# Autodesk Inventor assembly: PoweredWheelAssembly
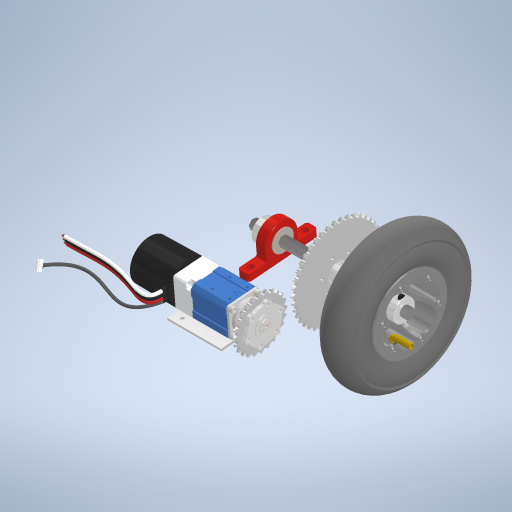
[picture p0: Inventor's stored thumbnail of the model, 512x512]
Saved by Autodesk Inventor 2023 (Build 270158000, 158)
## iProperties
Created: 2022-09-14
Part Number: PoweredWheelAssembly
Document SubType Name: Assembly
Designer: PC
Author: PC
## Documents named in this file (12)
- C:\Users\PC\Documents\PersonalCAD\ARCIGVC\IGVC-Robot\PoweredWheelAssembly.iam
- C:\Users\PC\Documents\PersonalCAD\ARCIGVC\IGVC-Robot\8inPneumatic.ipt
- C:\Users\PC\Documents\PersonalCAD\ARCIGVC\IGVC-Robot\2 Stage HD - CIM Sport.ipt
- C:\Users\PC\Documents\PersonalCAD\ARCIGVC\IGVC-Robot\am-4258 NEO Brushless Motor.ipt
- C:\Users\PC\Documents\PersonalCAD\ARCIGVC\IGVC-Robot\MotorMount.ipt
- C:\Users\PC\Documents\PersonalCAD\ARCIGVC\IGVC-Robot\24tSprocket35Series.ipt
- C:\Users\PC\Documents\PersonalCAD\ARCIGVC\IGVC-Robot\42tSprocket35Series.ipt
- C:\Users\PC\Documents\PersonalCAD\ARCIGVC\IGVC-Robot\Hex Hub .5In.ipt
- C:\Users\PC\Documents\PersonalCAD\ARCIGVC\IGVC-Robot\Bearing Housing.ipt
- C:\Users\PC\Documents\PersonalCAD\ARCIGVC\IGVC-Robot\HalfInHex Bearing.ipt
- C:\Users\PC\Documents\PersonalCAD\ARCIGVC\IGVC-Robot\9in-0.5inHexAxel.ipt
- C:\Users\PC\Documents\PersonalCAD\ARCIGVC\IGVC-Robot\am-1526 500Hex HD Collar Clamp.ipt
## Components (17 placed, 11 different names)
1. 8inPneumatic:1 — Mate:35
2. 2 Stage HD - CIM Sport:1
3. am-4258 NEO Brushless Motor:1
4. MotorMount:1 — Flush:6, Flush:7
5. 24tSprocket35Series:1
6. 42tSprocket35Series:1
7. Hex Hub .5In:1
8. Hex Hub .5In:2
9. Bearing Housing:1 — Flush:4, Mate:35
10. Bearing Housing:2 — Flush:4, Flush:5, Flush:6, Flush:7
11. HalfInHex Bearing:1
12. HalfInHex Bearing:2
13. HalfInHex Bearing:3
14. HalfInHex Bearing:4
15. 9in-0.5inHexAxel:1 — Flush:5
16. am-1526 500Hex HD Collar Clamp:1
17. am-1526 500Hex HD Collar Clamp:2
## Relationships (42: Mate 35, Flush 7)
- [Mate]: 2 Stage HD - CIM Sport:1 ↔ am-4258 NEO Brushless Motor:1
- [Mate]: 2 Stage HD - CIM Sport:1 ↔ am-4258 NEO Brushless Motor:1
- [Mate]: 2 Stage HD - CIM Sport:1 ↔ am-4258 NEO Brushless Motor:1
- [Mate]: 2 Stage HD - CIM Sport:1 ↔ MotorMount:1
- [Mate]: 2 Stage HD - CIM Sport:1 ↔ MotorMount:1
- [Mate]: 2 Stage HD - CIM Sport:1 ↔ MotorMount:1
- [Mate]: 24tSprocket35Series:1 ↔ Hex Hub .5In:2
- [Mate]: 24tSprocket35Series:1 ↔ Hex Hub .5In:2
- [Mate]: 24tSprocket35Series:1 ↔ Hex Hub .5In:2
- [Mate]: 2 Stage HD - CIM Sport:1 ↔ Hex Hub .5In:2
- [Flush]: 2 Stage HD - CIM Sport:1 ↔ Hex Hub .5In:2
- [Mate]: 42tSprocket35Series:1 ↔ Hex Hub .5In:1
- [Mate]: 42tSprocket35Series:1 ↔ Hex Hub .5In:1
- [Mate]: 42tSprocket35Series:1 ↔ Hex Hub .5In:1
- [Mate]: Bearing Housing:1 ↔ Bearing Housing:2
- [Mate]: Bearing Housing:1 ↔ HalfInHex Bearing:1
- [Mate]: Bearing Housing:1 ↔ HalfInHex Bearing:1
- [Mate]: Bearing Housing:1 ↔ HalfInHex Bearing:2
- [Mate]: Bearing Housing:1 ↔ HalfInHex Bearing:2
- [Mate]: Bearing Housing:2 ↔ HalfInHex Bearing:3
- [Mate]: Bearing Housing:2 ↔ HalfInHex Bearing:4
- [Mate]: Bearing Housing:2 ↔ HalfInHex Bearing:4
- [Mate]: Bearing Housing:2 ↔ HalfInHex Bearing:3
- [Mate]: 8inPneumatic:1 ↔ Bearing Housing:1
- [Mate]: Hex Hub .5In:1 ↔ Bearing Housing:1
- [Flush]: 24tSprocket35Series:1 ↔ 42tSprocket35Series:1
- [Mate]: Hex Hub .5In:1 ↔ 9in-0.5inHexAxel:1
- [Mate]: Hex Hub .5In:1 ↔ 9in-0.5inHexAxel:1
- [Flush]: 8inPneumatic:1 ↔ 9in-0.5inHexAxel:1
- [Mate]: 8inPneumatic:1 ↔ 9in-0.5inHexAxel:1
- [Mate]: 9in-0.5inHexAxel:1 ↔ am-1526 500Hex HD Collar Clamp:2
- [Mate]: 9in-0.5inHexAxel:1 ↔ am-1526 500Hex HD Collar Clamp:2
- [Mate] (25.4 mm): MotorMount:1 ↔ Bearing Housing:2
- [Mate]: HalfInHex Bearing:3 ↔ am-1526 500Hex HD Collar Clamp:2
- [Mate]: 9in-0.5inHexAxel:1 ↔ am-1526 500Hex HD Collar Clamp:1
- [Mate]: 9in-0.5inHexAxel:1 ↔ am-1526 500Hex HD Collar Clamp:1
- [Mate]: 8inPneumatic:1 ↔ am-1526 500Hex HD Collar Clamp:1
- Flush:4: Bearing Housing:1 ↔ Bearing Housing:2
- Mate:35 (17.4752 mm): 8inPneumatic:1 ↔ Bearing Housing:1
- Flush:5 (25.5778 mm): Bearing Housing:2 ↔ 9in-0.5inHexAxel:1
- Flush:6 (4.7752 mm): MotorMount:1 ↔ Bearing Housing:2
- Flush:7: MotorMount:1 ↔ Bearing Housing:2
